# Autodesk Inventor assembly: 001_ring
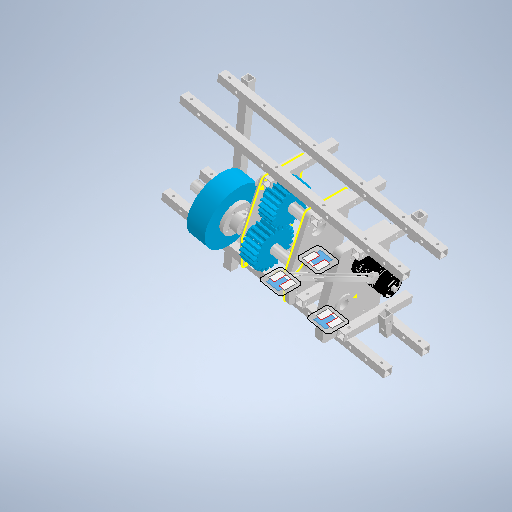
[picture p0: Inventor's stored thumbnail of the model, 512x512]
Saved by Autodesk Inventor 2025.1 (Build 291241000, 241)
## iProperties
Created: 2024-10-03
Part Number: 001_ring
Document SubType Name: Assembly
Designer: yuki0520
Author: yuki0520
## Documents named in this file (15)
- C:\Users\yuki0520\OneDrive\ドキュメント\Inventor\2025_nhk\tanaka\nageru\smallring\001_ring.iam
- C:\Users\yuki0520\OneDrive\ドキュメント\Inventor\2025_nhk\tanaka\nageru\pakuriz\kaku_1010_120.ipt
- C:\Users\yuki0520\OneDrive\ドキュメント\Inventor\2025_nhk\tanaka\nageru\pakuriz\bear_12_18.ipt
- C:\Users\yuki0520\OneDrive\ドキュメント\Inventor\2025_nhk\tanaka\nageru\smallring\small_tire.ipt
- C:\Users\yuki0520\OneDrive\ドキュメント\Inventor\2025_nhk\tanaka\nageru\smallring\small_tire_fixer.ipt
- C:\Users\yuki0520\OneDrive\ドキュメント\Inventor\2025_nhk\tanaka\nageru\smallring\small_bar_roller.ipt
- C:\Users\yuki0520\OneDrive\ドキュメント\Inventor\2025_nhk\tanaka\nageru\smallring\small_plate_motor.ipt
- C:\Users\yuki0520\OneDrive\ドキュメント\Inventor\2025_nhk\tanaka\nageru\smallring\small_plate_middle.ipt
- C:\Users\yuki0520\OneDrive\ドキュメント\Inventor\2025_nhk\tanaka\nageru\smallring\small_plate_nomotor.ipt
- C:\Users\yuki0520\OneDrive\ドキュメント\Inventor\2025_nhk\tanaka\nageru\smallring\small_gear_motor_48.iam
- C:\Users\yuki0520\OneDrive\ドキュメント\Inventor\2025_nhk\tanaka\nageru\smallring\small_kaku_1010_bridge.ipt
- C:\Users\yuki0520\OneDrive\ドキュメント\Inventor\2025_nhk\tanaka\nageru\smallring\small_kaku_1010_santen.ipt
- C:\Users\yuki0520\OneDrive\ドキュメント\Inventor\2025_nhk\tanaka\nageru\smallring\small_kaku_1010_200.ipt
- C:\Users\yuki0520\OneDrive\ドキュメント\Inventor\2025_nhk\tanaka\nageru\smallring\small_bar_motor.ipt
- C:\Users\yuki0520\OneDrive\ドキュメント\Inventor\2025_nhk\tanaka\nageru\inventorパーツリスト\モーター\RoboMaster M2006 P36.ipt
## Components (27 placed, 14 different names)
1. kaku_1010_120:1 — 挿入:83, 挿入:89, メイト:78, 挿入:112, 挿入:126
2. kaku_1010_120:2 — 挿入:86, 挿入:92, 挿入:130, 挿入:131
3. kaku_1010_120:3 — 挿入:81, 挿入:87, メイト:79, フラッシュ:1, 挿入:118, 挿入:127
4. kaku_1010_120:4 — 挿入:91, 挿入:128, 挿入:129
5. bear_12_18:1 — メイト:33, メイト:37
6. bear_12_18:2 — メイト:35, メイト:36
7. kaku_1010_120:5 — 挿入:82, 挿入:88, 挿入:115, 挿入:125
8. kaku_1010_120:6 — 挿入:95, 挿入:132, 挿入:133
9. small_tire:1 — メイト:8, 挿入:97, 挿入:98
10. small_tire_fixer:1 — メイト:9, メイト:95
11. small_bar_roller:1 — メイト:8, メイト:9, メイト:26, メイト:27, メイト:30, メイト:33, メイト:35, メイト:38, メイト:88, メイト:95, メイト:96
12. small_plate_motor:1 — メイト:26, メイト:36, メイト:78, 挿入:112, 挿入:123, 挿入:124, 挿入:126, 挿入:132, 挿入:133
13. small_plate_middle:1 — メイト:102, 挿入:115, メイト:104, 挿入:125, 挿入:128, 挿入:129
14. small_plate_nomotor:1 — メイト:37, メイト:79, メイト:96, 挿入:118, 挿入:127, 挿入:130, 挿入:131
15. small_gear_motor_48:1 [sub-assembly] — メイト:27, メイト:38, メイト:94
16. small_tire_fixer:2 — メイト:30, 挿入:97, 挿入:98
17. small_kaku_1010_bridge:1 — 挿入:121
18. small_kaku_1010_santen:1 — 挿入:95
19. small_kaku_1010_santen:2 — 挿入:71
20. small_kaku_1010_200:1 — 挿入:71, 挿入:81, 挿入:82, 挿入:83, 挿入:121
21. small_kaku_1010_200:2 — 挿入:87, 挿入:88, 挿入:89
22. small_kaku_1010_200:3 — 挿入:91, 挿入:92
23. small_kaku_1010_200:4 — 挿入:86
24. bear_12_18:4 — メイト:88
25. small_bar_motor:1 — メイト:94, メイト:103
26. bear_12_18:6 — メイト:102, メイト:103, メイト:104
27. RoboMaster M2006 P36:1 — 挿入:123, 挿入:124
## Relationships (48: Insert 28, Mate 19, Flush 1)
- メイト:8 [Mate]: small_tire:1 ↔ small_bar_roller:1
- メイト:9 [Mate]: small_tire_fixer:1 ↔ small_bar_roller:1
- メイト:26 [Mate]: small_bar_roller:1 ↔ small_plate_motor:1
- メイト:27 [Mate]: small_bar_roller:1 ↔ small_gear_motor_48:1
- メイト:30 [Mate]: small_bar_roller:1 ↔ small_tire_fixer:2
- メイト:33 [Mate]: bear_12_18:1 ↔ small_bar_roller:1
- メイト:35 [Mate]: bear_12_18:2 ↔ small_bar_roller:1
- メイト:36 [Mate]: bear_12_18:2 ↔ small_plate_motor:1
- メイト:37 [Mate]: bear_12_18:1 ↔ small_plate_nomotor:1
- メイト:38 [Mate]: small_bar_roller:1 ↔ small_gear_motor_48:1
- 挿入:71 [Insert]: small_kaku_1010_santen:2 ↔ small_kaku_1010_200:1
- 挿入:81 [Insert]: kaku_1010_120:3 ↔ small_kaku_1010_200:1
- 挿入:82 [Insert]: kaku_1010_120:5 ↔ small_kaku_1010_200:1
- 挿入:83 [Insert]: kaku_1010_120:1 ↔ small_kaku_1010_200:1
- 挿入:86 [Insert]: kaku_1010_120:2 ↔ small_kaku_1010_200:4
- 挿入:87 [Insert]: kaku_1010_120:3 ↔ small_kaku_1010_200:2
- 挿入:88 [Insert]: kaku_1010_120:5 ↔ small_kaku_1010_200:2
- 挿入:89 [Insert]: kaku_1010_120:1 ↔ small_kaku_1010_200:2
- 挿入:91 [Insert]: kaku_1010_120:4 ↔ small_kaku_1010_200:3
- 挿入:92 [Insert]: kaku_1010_120:2 ↔ small_kaku_1010_200:3
- メイト:78 [Mate]: kaku_1010_120:1 ↔ small_plate_motor:1
- メイト:79 [Mate]: kaku_1010_120:3 ↔ small_plate_nomotor:1
- 挿入:95 [Insert]: kaku_1010_120:6 ↔ small_kaku_1010_santen:1
- メイト:88 [Mate]: small_bar_roller:1 ↔ bear_12_18:4
- メイト:94 [Mate]: small_gear_motor_48:1 ↔ small_bar_motor:1
- フラッシュ:1 [Flush]: kaku_1010_120:3
- 挿入:97 [Insert]: small_tire:1 ↔ small_tire_fixer:2
- 挿入:98 [Insert]: small_tire:1 ↔ small_tire_fixer:2
- メイト:95 [Mate]: small_tire_fixer:1 ↔ small_bar_roller:1
- メイト:96 [Mate]: small_bar_roller:1 ↔ small_plate_nomotor:1
- メイト:102 [Mate]: small_plate_middle:1 ↔ bear_12_18:6
- 挿入:112 [Insert]: kaku_1010_120:1 ↔ small_plate_motor:1
- 挿入:115 [Insert]: kaku_1010_120:5 ↔ small_plate_middle:1
- 挿入:118 [Insert]: kaku_1010_120:3 ↔ small_plate_nomotor:1
- 挿入:121 [Insert]: small_kaku_1010_bridge:1 ↔ small_kaku_1010_200:1
- メイト:103 [Mate]: small_bar_motor:1 ↔ bear_12_18:6
- メイト:104 [Mate]: small_plate_middle:1 ↔ bear_12_18:6
- 挿入:123 [Insert]: small_plate_motor:1 ↔ RoboMaster M2006 P36:1
- 挿入:124 [Insert]: small_plate_motor:1 ↔ RoboMaster M2006 P36:1
- 挿入:125 [Insert]: kaku_1010_120:5 ↔ small_plate_middle:1
- 挿入:126 [Insert]: kaku_1010_120:1 ↔ small_plate_motor:1
- 挿入:127 [Insert]: kaku_1010_120:3 ↔ small_plate_nomotor:1
- 挿入:128 [Insert]: kaku_1010_120:4 ↔ small_plate_middle:1
- 挿入:129 [Insert]: kaku_1010_120:4 ↔ small_plate_middle:1
- 挿入:130 [Insert]: kaku_1010_120:2 ↔ small_plate_nomotor:1
- 挿入:131 [Insert]: kaku_1010_120:2 ↔ small_plate_nomotor:1
- 挿入:132 [Insert]: kaku_1010_120:6 ↔ small_plate_motor:1
- 挿入:133 [Insert]: kaku_1010_120:6 ↔ small_plate_motor:1
